# Autodesk Inventor assembly: uMule-Koło
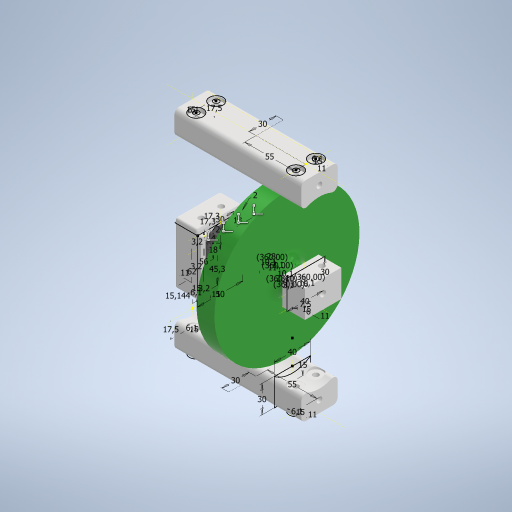
[picture p0: Inventor's stored thumbnail of the model, 512x512]
Saved by Autodesk Inventor 2024.3 (Build 283343000, 343)
## iProperties
Created: 2024-10-21
Part Number: uMule-Koło
Document SubType Name: Assembly
Designer: owozn
Author: owozn
## Documents named in this file (6)
- C:\Users\owozn\Documents\Nauka\Studia\mgr\Semestr_3\Magisterka\temp\uMule\mechanics\uMule-Koło.iam
- C:\Users\owozn\Documents\Nauka\Studia\mgr\Semestr_3\Magisterka\temp\uMule\mechanics\uMule-kolo_napędowe.ipt
- C:\Users\owozn\Documents\Nauka\Studia\mgr\Semestr_3\Magisterka\temp\uMule\mechanics\rx64H\rx64H.ipt
- C:\Users\owozn\Documents\Nauka\Studia\mgr\Semestr_3\Magisterka\temp\uMule\mechanics\uMule-Uchwyt_koła.ipt
- C:\Users\owozn\Documents\Nauka\Studia\mgr\Semestr_3\Magisterka\temp\uMule\mechanics\uMule-ogranicznik_koła.ipt
- C:\Users\owozn\Documents\Nauka\Studia\mgr\Semestr_3\Magisterka\temp\uMule\mechanics\uMule-uchwyt_dx_góra.ipt
## Components (7 placed, 5 different names)
1. uMule-kolo_napędowe:1 — Mate:1, Mate:2, Mate:3, Mate:4, Mate:7
2. uMule-kolo_napędowe:2 — Mate:1, Mate:2, Mate:3, Mate:5
3. rx64H:1 — Mate:4, Mate:5, Flush:2, Mate:15, Mate:16
4. uMule-Uchwyt_koła:1 — Mate:7, Mate:10, Flush:3, Flush:4
5. uMule-ogranicznik_koła:1 — Mate:10, Mate:11, Mate:12, Flush:4, Flush:6
6. uMule-ogranicznik_koła:2 — Mate:11, Mate:12, Flush:3, Flush:5, Flush:6
7. uMule-uchwyt_dx_góra:1 — Flush:2, Mate:15, Mate:16, Flush:5
## Relationships (16: Mate 11, Flush 5)
- Mate:1: uMule-kolo_napędowe:1 ↔ uMule-kolo_napędowe:2
- Mate:2: uMule-kolo_napędowe:1 ↔ uMule-kolo_napędowe:2
- Mate:3: uMule-kolo_napędowe:1 ↔ uMule-kolo_napędowe:2
- Mate:4: uMule-kolo_napędowe:1 ↔ rx64H:1
- Mate:5: uMule-kolo_napędowe:2 ↔ rx64H:1
- Mate:7 (4 mm): uMule-kolo_napędowe:1 ↔ uMule-Uchwyt_koła:1
- Mate:10: uMule-Uchwyt_koła:1 ↔ uMule-ogranicznik_koła:1
- Mate:11: uMule-ogranicznik_koła:1 ↔ uMule-ogranicznik_koła:2
- Mate:12: uMule-ogranicznik_koła:1 ↔ uMule-ogranicznik_koła:2
- Flush:2: rx64H:1 ↔ uMule-uchwyt_dx_góra:1
- Mate:15: rx64H:1 ↔ uMule-uchwyt_dx_góra:1
- Mate:16: rx64H:1 ↔ uMule-uchwyt_dx_góra:1
- Flush:3 (100 mm): uMule-Uchwyt_koła:1 ↔ uMule-ogranicznik_koła:2
- Flush:4 (100 mm): uMule-Uchwyt_koła:1 ↔ uMule-ogranicznik_koła:1
- Flush:5 (5 mm): uMule-ogranicznik_koła:2 ↔ uMule-uchwyt_dx_góra:1
- Flush:6: uMule-ogranicznik_koła:1 ↔ uMule-ogranicznik_koła:2
